# Autodesk Inventor assembly: elbow
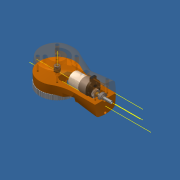
[picture p0: Inventor's stored thumbnail of the model, 180x180]
Saved by Autodesk Inventor 2014 SP2 (Build 180246200, 246)
## iProperties
Created: 2015-01-18
Part Number: elbow
Document SubType Name: Assembly
Designer: 4ndreas
Author: 4ndreas
## Documents named in this file (20)
- C:\Users\4ndreas\Documents\Inventor\RobotARM v2\v2\elbow.iam
- C:\Users\4ndreas\Documents\Inventor\RobotARM v2\ArmSegment_klein.ipt
- C:\Users\4ndreas\Documents\Inventor\RobotARM v2\v2\conrad_getriebe_motor.ipt
- C:\Users\4ndreas\Documents\Inventor\RobotARM v2\rotRohr.ipt
- C:\Users\4ndreas\Documents\Inventor\Content Center Files\R2014\de-DE\DIN BEARING(1)\DIN 625 SKF - SKF 608.ipt
- C:\Users\4ndreas\Documents\Inventor\RobotARM v2\v2\elbowMotorHolder.ipt
- C:\Users\4ndreas\Documents\Inventor\RobotARM v2\v2\FaulhaberMotor.ipt
- C:\Users\4ndreas\Documents\Inventor\RobotARM v2\v2\ArmSegment_klein_Gear.ipt
- C:\Users\4ndreas\Documents\Inventor\Content Center Files\R2014\de-DE\DIN 985\DIN 985 - M8.ipt
- C:\Users\4ndreas\Documents\Inventor\RobotARM v2\v2\elbow\Konstruktions-Assistent\Übertragung des Zahnriemens1.iam
- C:\Users\4ndreas\Documents\Inventor\RobotARM v2\Nema17 Geared.ipt
- C:\Users\4ndreas\Documents\Inventor\RobotARM v2\v2\DIN 625 SKF - SKF 618_5_5mm.ipt
- C:\Users\4ndreas\Documents\Inventor\RobotARM v2\v2\elbow\Konstruktions-Assistent\Stirnräder2.iam
- C:\Users\4ndreas\Documents\Inventor\Content Center Files\R2014\de-DE\DIN 931-1\DIN 931-1 - M5 x 25.ipt
- C:\Users\4ndreas\Documents\Inventor\Content Center Files\R2014\de-DE\DIN 985\DIN 985 - M5.ipt
- C:\Users\4ndreas\Documents\Inventor\Content Center Files\R2014\de-DE\DIN 433-1  A\DIN 433 - 5,3.ipt
- C:\Users\4ndreas\Documents\Inventor\RobotARM v2\v2\messingnut.ipt
- C:\Users\4ndreas\Documents\Inventor\RobotARM v2\v2\minimalEncoder.ipt
- C:\Users\4ndreas\Documents\Inventor\RobotARM v2\v2\Nutspacker.ipt
- C:\Users\4ndreas\Documents\Inventor\RobotARM v2\v2\M5_encoderMagnet.ipt
## Components (21 placed, 19 different names)
1. ArmSegment_klein:1 — Passend:1, Winkel:1, Winkel:2, Fluchtend:1, Passend:15, Passend:16, Fluchtend:2, Passend:17, Passend:20, Passend:21, Passend:50
2. ArmSegment_klein_Gear:1 — Passend:16, Fluchtend:2, Passend:17, Passend:18, Passend:19, Winkel:3, Passend:24
3. elbowMotorHolder:1 — Passend:14, Passend:15, Passend:30, Passend:33, Passend:34, Fluchtend:6
4. conrad_getriebe_motor:1 — Passend:2, Passend:4, Passend:5, Passend:6, Passend:10, Passend:12, Fluchtend:4
5. rotRohr:1 — Passend:9, Passend:10, Passend:11
6. DIN 625 SKF 608:1 — Passend:11, Fluchtend:1, Passend:12
7. FaulhaberMotor:1 — Passend:13, Passend:14
8. DIN 985 - ersetzt durch DIN EN ISO 10511 M8:2 — Passend:18, Passend:19
9. DIN 985 - ersetzt durch DIN EN ISO 10511 M8:3 — Passend:20, Passend:21
10. Übertragung des Zahnriemens:1 [sub-assembly] — Passend:29
11. Nema17 Geared:1 — Passend:29, Passend:30, Winkel:4
12. DIN 625 SKF 618/5:1 — Passend:34, Passend:36
13. DIN 625 SKF 618/5:2 — Passend:33, Passend:35, Passend:46
14. Stirnräder:1 [sub-assembly] — Passend:37, Fluchtend:4, Passend:38, Passend:42, Passend:44, Fluchtend:5, Passend:45
15. DIN 931-1 - ersetzt durch DIN EN 24014 M5 x 25:1 — Passend:39, Passend:40, Passend:41, Winkel:5, Passend:46, Passend:47, Passend:48, Passend:49
16. DIN 985 - ersetzt durch DIN EN ISO 10511 M5:1 — Passend:41, Winkel:5, Passend:42, Passend:45
17. DIN 433-1 A 5,3:1 — Passend:40
18. messingnut:1 — Passend:43, Passend:44, Fluchtend:5
19. minimalEncoder:1 — Passend:47
20. Nutspacker:1
21. M5_encoderMagnet:1 — Passend:48, Passend:49
## Relationships (55: Mate 44, Flush 6, Angle 5)
- Passend:1 [Mate]: ArmSegment_klein:1
- Winkel:1 [Angle] (0 deg): ArmSegment_klein:1
- Passend:2 [Mate]: conrad_getriebe_motor:1
- Passend:3 [Mate]
- Passend:4 [Mate]: conrad_getriebe_motor:1
- Passend:5 [Mate]: conrad_getriebe_motor:1
- Passend:6 [Mate]: conrad_getriebe_motor:1
- Passend:7 [Mate]
- Passend:8 [Mate]
- Winkel:2 [Angle] (0 deg): ArmSegment_klein:1
- Passend:9 [Mate]: rotRohr:1
- Passend:10 [Mate] (1 mm): conrad_getriebe_motor:1 ↔ rotRohr:1
- Passend:11 [Mate]: rotRohr:1 ↔ DIN 625 SKF 608:1
- Fluchtend:1 [Flush] (-5 mm): ArmSegment_klein:1 ↔ DIN 625 SKF 608:1
- Passend:12 [Mate] (6 mm): conrad_getriebe_motor:1 ↔ DIN 625 SKF 608:1
- Passend:13 [Mate]: FaulhaberMotor:1
- Passend:14 [Mate]: elbowMotorHolder:1 ↔ FaulhaberMotor:1
- Passend:15 [Mate]: ArmSegment_klein:1 ↔ elbowMotorHolder:1
- Passend:16 [Mate]: ArmSegment_klein:1 ↔ ArmSegment_klein_Gear:1
- Fluchtend:2 [Flush]: ArmSegment_klein:1 ↔ ArmSegment_klein_Gear:1
- Passend:17 [Mate]: ArmSegment_klein:1 ↔ ArmSegment_klein_Gear:1
- Passend:18 [Mate]: ArmSegment_klein_Gear:1 ↔ DIN 985 - ersetzt durch DIN EN ISO 10511 M8:2
- Passend:19 [Mate]: ArmSegment_klein_Gear:1 ↔ DIN 985 - ersetzt durch DIN EN ISO 10511 M8:2
- Passend:20 [Mate]: ArmSegment_klein:1 ↔ DIN 985 - ersetzt durch DIN EN ISO 10511 M8:3
- Passend:21 [Mate]: ArmSegment_klein:1 ↔ DIN 985 - ersetzt durch DIN EN ISO 10511 M8:3
- Passend:22 [Mate]
- Winkel:3 [Angle] (90 deg): ArmSegment_klein_Gear:1
- Fluchtend:3 [Flush] (18 mm)
- Passend:23 [Mate]
- Passend:24 [Mate]: ArmSegment_klein_Gear:1
- Passend:29 [Mate]: Übertragung des Zahnriemens:1 ↔ Nema17 Geared:1
- Passend:30 [Mate]: elbowMotorHolder:1 ↔ Nema17 Geared:1
- Winkel:4 [Angle] (0 deg): Nema17 Geared:1
- Passend:33 [Mate]: elbowMotorHolder:1 ↔ DIN 625 SKF 618/5:2
- Passend:34 [Mate]: elbowMotorHolder:1 ↔ DIN 625 SKF 618/5:1
- Passend:35 [Mate]: DIN 625 SKF 618/5:2
- Passend:36 [Mate]: DIN 625 SKF 618/5:1
- Passend:37 [Mate]: Stirnräder:1
- Fluchtend:4 [Flush] (-7 mm): conrad_getriebe_motor:1 ↔ Stirnräder:1
- Passend:38 [Mate]: Stirnräder:1
- Passend:39 [Mate]: DIN 931-1 - ersetzt durch DIN EN 24014 M5 x 25:1
- Passend:40 [Mate]: DIN 931-1 - ersetzt durch DIN EN 24014 M5 x 25:1 ↔ DIN 433-1 A 5,3:1
- Passend:41 [Mate]: DIN 931-1 - ersetzt durch DIN EN 24014 M5 x 25:1 ↔ DIN 985 - ersetzt durch DIN EN ISO 10511 M5:1
- Winkel:5 [Angle] (0 deg): DIN 931-1 - ersetzt durch DIN EN 24014 M5 x 25:1 ↔ DIN 985 - ersetzt durch DIN EN ISO 10511 M5:1
- Passend:42 [Mate]: Stirnräder:1 ↔ DIN 985 - ersetzt durch DIN EN ISO 10511 M5:1
- Passend:43 [Mate]: messingnut:1
- Passend:44 [Mate]: Stirnräder:1 ↔ messingnut:1
- Fluchtend:5 [Flush]: Stirnräder:1 ↔ messingnut:1
- Passend:45 [Mate]: Stirnräder:1 ↔ DIN 985 - ersetzt durch DIN EN ISO 10511 M5:1
- Passend:46 [Mate]: DIN 625 SKF 618/5:2 ↔ DIN 931-1 - ersetzt durch DIN EN 24014 M5 x 25:1
- Fluchtend:6 [Flush] (8 mm): elbowMotorHolder:1
- Passend:47 [Mate] (5 mm): DIN 931-1 - ersetzt durch DIN EN 24014 M5 x 25:1 ↔ minimalEncoder:1
- Passend:48 [Mate]: DIN 931-1 - ersetzt durch DIN EN 24014 M5 x 25:1 ↔ M5_encoderMagnet:1
- Passend:49 [Mate]: DIN 931-1 - ersetzt durch DIN EN 24014 M5 x 25:1 ↔ M5_encoderMagnet:1
- Passend:50 [Mate]: ArmSegment_klein:1
